# Autodesk Inventor assembly: 1stLayout
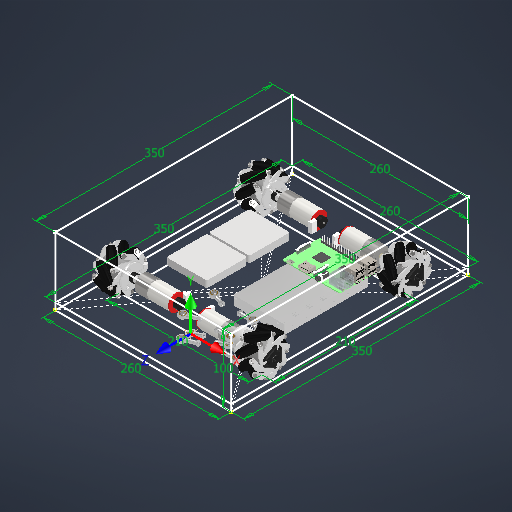
[picture p0: Inventor's stored thumbnail of the model, 512x512]
Saved by Autodesk Inventor 2025 (Build 290162000, 162)
## iProperties
Created: 2024-10-02
Part Number: 1stLayout
Document SubType Name: Assembly
Designer: khrip
Author: khrip
## Documents named in this file (11)
- H:\Potamon\3Dmodels\Chassis\1stLayout.iam
- H:\Potamon\3Dmodels\UnsprungUnits\Wheels\wheel assembly.iam
- H:\Potamon\3Dmodels\UnsprungUnits\Wheels\wheel assemblyMirrored.iam
- H:\Potamon\3Dmodels\UnsprungUnits\Parts\servo.ipt
- H:\Potamon\3Dmodels\Chassis\MaxDimensions.ipt
- H:\Potamon\3Dmodels\Chassis\Parts\ServocontrollerSizer.ipt
- H:\Potamon\3Dmodels\Parts\raspberry\RaspberryPi2 STEP214.iam
- H:\Potamon\3Dmodels\Parts\18650_X6.ipt
- C:\Users\khrip\Documents\Inventor\Content Center Files\R2025\ru-RU\JIS B 1521\JIS B 1521 - 6801 12x21x5x1,92.ipt
- H:\Potamon\3Dmodels\UnsprungUnits\Parts\Knuckle.ipt
- H:\Potamon\3Dmodels\BallJoint3mm\BallJoint3mm.iam
## Components (27 placed, 10 different names)
1. wheel assembly:1 [sub-assembly] — Заподлицо:2, Совмещение:1, Заподлицо:3, Совмещение:10, Совмещение:15, Совмещение:21, Совмещение:22
2. wheel assemblyMirrored:1 [sub-assembly] — Заподлицо:1, Совмещение:2, Заподлицо:4, Совмещение:9, Совмещение:14, Совмещение:19, Совмещение:20
3. wheel assembly:2 [sub-assembly] — Совмещение:4, Совмещение:5, Совмещение:8, Совмещение:12, Совмещение:13, Совмещение:17, Совмещение:18, Заподлицо:6
4. wheel assemblyMirrored:2 [sub-assembly] — Совмещение:3, Совмещение:6, Совмещение:7, Совмещение:11, Совмещение:16, Совмещение:23, Совмещение:24
5. servo:1 — Угол:1, Совмещение:9, Совмещение:14
6. servo:2 — Угол:2, Совмещение:10, Совмещение:15
7. servo:3 — Угол:3, Совмещение:11, Совмещение:16
8. servo:4 — Угол:4, Совмещение:12, Совмещение:13, Заподлицо:7
9. MaxDimensions:1 — Заподлицо:5
10. ServocontrollerSizer:1
11. ServocontrollerSizer:2
12. RaspberryPi2 STEP214:1 [sub-assembly]
13. 18650_X6:1 — Угол:5, Угол:6
14. JIS B 1521 6801 12x21x5:1 — Совмещение:17, Совмещение:18
15. JIS B 1521 6801 12x21x5:2 — Совмещение:19, Совмещение:20
16. JIS B 1521 6801 12x21x5:3 — Совмещение:21, Совмещение:22
17. JIS B 1521 6801 12x21x5:4 — Совмещение:23, Совмещение:24
18. Knuckle:1 — Заподлицо:6, Заподлицо:7
19. BallJoint3mm:1 [sub-assembly]
20. BallJoint3mm:2 [sub-assembly]
21. BallJoint3mm:3 [sub-assembly]
22. BallJoint3mm:4 [sub-assembly]
23. BallJoint3mm:5 [sub-assembly]
24. BallJoint3mm:6 [sub-assembly]
25. BallJoint3mm:7 [sub-assembly]
26. BallJoint3mm:8 [sub-assembly]
27. BallJoint3mm:9 [sub-assembly]
## Relationships (37: Mate 24, Flush 7, Angle 6)
- Заподлицо:1 [Flush] (105 mm): wheel assemblyMirrored:1
- Заподлицо:2 [Flush] (105 mm): wheel assembly:1
- Совмещение:1 [Mate] (30 mm): wheel assembly:1
- Совмещение:2 [Mate] (30 mm): wheel assemblyMirrored:1
- Заподлицо:3 [Flush] (105 mm): wheel assembly:1
- Заподлицо:4 [Flush] (-105 mm): wheel assemblyMirrored:1
- Совмещение:3 [Mate] (105 mm): wheel assemblyMirrored:2
- Совмещение:4 [Mate] (105 mm): wheel assembly:2
- Совмещение:5 [Mate] (30 mm): wheel assembly:2
- Совмещение:6 [Mate] (30 mm): wheel assemblyMirrored:2
- Совмещение:7 [Mate] (-105 mm): wheel assemblyMirrored:2
- Совмещение:8 [Mate] (105 mm): wheel assembly:2
- Угол:1 [Angle] (180 deg): servo:1
- Совмещение:9 [Mate]: wheel assemblyMirrored:1 ↔ servo:1
- Угол:2 [Angle] (0 deg): servo:2
- Совмещение:10 [Mate]: wheel assembly:1 ↔ servo:2
- Угол:3 [Angle] (0 deg): servo:3
- Совмещение:11 [Mate]: wheel assemblyMirrored:2 ↔ servo:3
- Угол:4 [Angle] (180 deg): servo:4
- Совмещение:12 [Mate]: wheel assembly:2 ↔ servo:4
- Заподлицо:5 [Flush]: MaxDimensions:1
- Угол:5 [Angle] (180 deg): 18650_X6:1
- Угол:6 [Angle] (0 deg): 18650_X6:1
- Совмещение:13 [Mate] (0.5 mm): wheel assembly:2 ↔ servo:4
- Совмещение:14 [Mate] (0.5 mm): wheel assemblyMirrored:1 ↔ servo:1
- Совмещение:15 [Mate] (0.5 mm): wheel assembly:1 ↔ servo:2
- Совмещение:16 [Mate] (0.5 mm): wheel assemblyMirrored:2 ↔ servo:3
- Совмещение:17 [Mate]: wheel assembly:2 ↔ JIS B 1521 6801 12x21x5:1
- Совмещение:18 [Mate]: wheel assembly:2 ↔ JIS B 1521 6801 12x21x5:1
- Совмещение:19 [Mate]: wheel assemblyMirrored:1 ↔ JIS B 1521 6801 12x21x5:2
- Совмещение:20 [Mate]: wheel assemblyMirrored:1 ↔ JIS B 1521 6801 12x21x5:2
- Совмещение:21 [Mate]: wheel assembly:1 ↔ JIS B 1521 6801 12x21x5:3
- Совмещение:22 [Mate]: wheel assembly:1 ↔ JIS B 1521 6801 12x21x5:3
- Совмещение:23 [Mate]: wheel assemblyMirrored:2 ↔ JIS B 1521 6801 12x21x5:4
- Совмещение:24 [Mate]: wheel assemblyMirrored:2 ↔ JIS B 1521 6801 12x21x5:4
- Заподлицо:6 [Flush]: wheel assembly:2 ↔ Knuckle:1
- Заподлицо:7 [Flush]: servo:4 ↔ Knuckle:1
